# Autodesk Inventor assembly: EvelbACKBeam
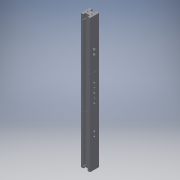
[picture p0: Inventor's stored thumbnail of the model, 180x180]
Saved by Autodesk Inventor 2019 (Build 230136000, 136)
## iProperties
Created: 2019-10-01
Part Number: EvelbACKBeam
Document SubType Name: Assembly
Designer: james
Author: james
## Documents named in this file (3)
- F:\JimsDesign\Jims2020FTC\EvelBackBeam.iam
- F:\JimsDesign\Library\McMaster\Screws\91771A152_18-8 SS FLAT HEAD PHILLIPS MACHINE SCREW.ipt
- F:\JimsDesign\Jims2020FTC\bACKBeamSplit.ipt
## Components (7 placed, 2 different names)
1. bACKBeamSplit:1 — Mate:1, Mate:2, Mate:3, Mate:4, Mate:5, Mate:6, Flush:3, Flush:4, Flush:5
2. bACKBeamSplit:2 — Mate:1, Mate:2, Mate:3, Mate:7, Mate:8, Flush:1, Flush:2
3. 91771A152_18-8 SS FLAT HEAD PHILLIPS MACHINE SCREW:1 — Mate:4, Flush:3
4. 91771A152_18-8 SS FLAT HEAD PHILLIPS MACHINE SCREW:2 — Mate:5, Flush:4
5. 91771A152_18-8 SS FLAT HEAD PHILLIPS MACHINE SCREW:3 — Mate:6, Flush:5
6. 91771A152_18-8 SS FLAT HEAD PHILLIPS MACHINE SCREW:4 — Mate:7, Flush:1
7. 91771A152_18-8 SS FLAT HEAD PHILLIPS MACHINE SCREW:5 — Mate:8, Flush:2
## Relationships (13: Mate 8, Flush 5)
- Mate:1: bACKBeamSplit:1 ↔ bACKBeamSplit:2
- Mate:2: bACKBeamSplit:1 ↔ bACKBeamSplit:2
- Mate:3: bACKBeamSplit:1 ↔ bACKBeamSplit:2
- Mate:4: bACKBeamSplit:1 ↔ 91771A152_18-8 SS FLAT HEAD PHILLIPS MACHINE SCREW:1
- Mate:5: bACKBeamSplit:1 ↔ 91771A152_18-8 SS FLAT HEAD PHILLIPS MACHINE SCREW:2
- Mate:6: bACKBeamSplit:1 ↔ 91771A152_18-8 SS FLAT HEAD PHILLIPS MACHINE SCREW:3
- Mate:7: bACKBeamSplit:2 ↔ 91771A152_18-8 SS FLAT HEAD PHILLIPS MACHINE SCREW:4
- Mate:8: bACKBeamSplit:2 ↔ 91771A152_18-8 SS FLAT HEAD PHILLIPS MACHINE SCREW:5
- Flush:1: bACKBeamSplit:2 ↔ 91771A152_18-8 SS FLAT HEAD PHILLIPS MACHINE SCREW:4
- Flush:2: bACKBeamSplit:2 ↔ 91771A152_18-8 SS FLAT HEAD PHILLIPS MACHINE SCREW:5
- Flush:3: bACKBeamSplit:1 ↔ 91771A152_18-8 SS FLAT HEAD PHILLIPS MACHINE SCREW:1
- Flush:4: bACKBeamSplit:1 ↔ 91771A152_18-8 SS FLAT HEAD PHILLIPS MACHINE SCREW:2
- Flush:5: bACKBeamSplit:1 ↔ 91771A152_18-8 SS FLAT HEAD PHILLIPS MACHINE SCREW:3
